# Autodesk Inventor assembly: HINGE-HENGZHU-40X40
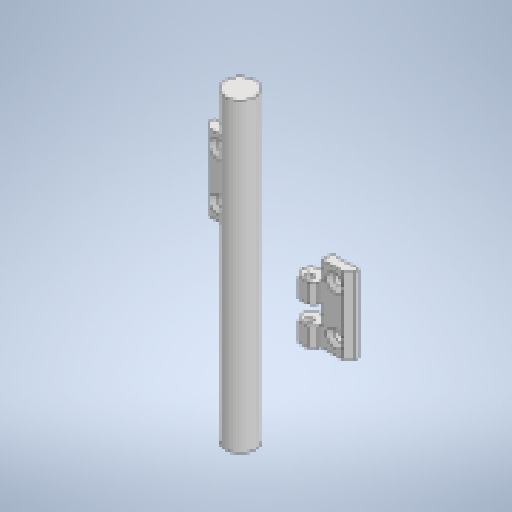
[picture p0: Inventor's stored thumbnail of the model, 512x512]
Saved by Autodesk Inventor 2024.3 (Build 283343000, 343)
## iProperties
Created: 2024-11-20
Part Number: HINGE-HENGZHU-40X40
Description: STEP AP203
Document SubType Name: Assembly
Designer: megha
Sending System: SolidWorks 2024
Preprocessor: SwSTEP 2.0
Title: HINGE-HENGZHU-40X40.STEP
Revision Number: ANY
## Documents named in this file (3)
- C:\Users\megha\KiCad\8.99\projects\delorean\CAD\HL050-2\HL050-2\HL050-2\HL050-2.iam
- C:\Users\megha\KiCad\8.99\projects\delorean\CAD\HL050-2\HL050-2\HL050-2\HINGE-HENGZHU-40X40-A1.ipt
- C:\Users\megha\KiCad\8.99\projects\delorean\CAD\HL050-2\HL050-2\HL050-2\Part24^Assem2.ipt
## Components (2 placed, 2 different names)
1. HINGE-HENGZHU-40X40-A1_1 — Mate:1
2. Part24^Assem2_3 — Mate:1
## Relationships (1: Mate 1)
- Mate:1: HINGE-HENGZHU-40X40-A1_1 ↔ Part24^Assem2_3
